# Autodesk Inventor assembly: Framing_For_Second_Floor
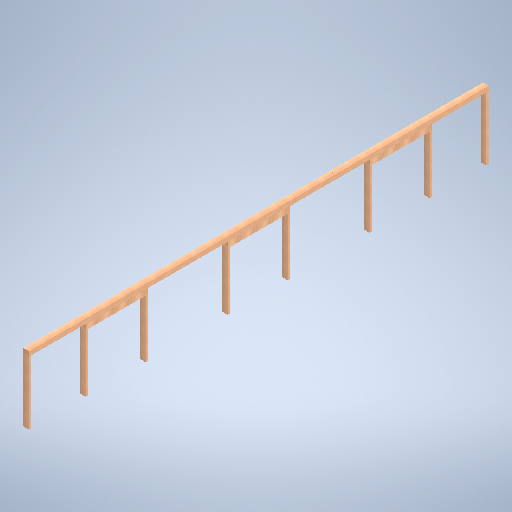
[picture p0: Inventor's stored thumbnail of the model, 512x512]
Saved by Autodesk Inventor 2025.1 (Build 291241020, 241B)
## iProperties
Created: 2024-10-21
Part Number: Framing_For_Second_Floor
Document SubType Name: Assembly
Designer: Tom
Author: Tom
## Documents named in this file (5)
- C:\Users\Tom\Documents\Inventor\Mobility\Additional_Building\Framing_For_Second_Floor.iam
- C:\Users\Tom\Documents\Inventor\Mobility\Additional_Building\Plate_With_Length_144_Inches.ipt
- C:\Users\Tom\Documents\Inventor\Mobility\Additional_Building\Plate_With_Length_96_Inches.ipt
- C:\Users\Tom\Documents\Inventor\Mobility\Additional_Building\Framing_For_Second_Floor_Window.iam
- C:\Users\Tom\Documents\Inventor\Mobility\Additional_Building\Stud_With_Height_39.5_Inches.ipt
## Components (10 placed, 4 different names)
1. Plate_With_Length_144_Inches:1 — Mate:2, Flush:3, Flush:4, Mate:3, Flush:5, Mate:4, Flush:7, Mate:9, Flush:9, Mate:12, Flush:11, Flush:12, Flush:15, Flush:16
2. Plate_With_Length_144_Inches:2 — Mate:2, Flush:3, Flush:4, Flush:6, Mate:6, Flush:8, Mate:11, Flush:10, Flush:17, Mate:13
3. Plate_With_Length_96_Inches:1 — Mate:3, Flush:5, Flush:6, Mate:5, Mate:7
4. Plate_With_Length_96_Inches:2 — Mate:4, Flush:7, Mate:5
5. Plate_With_Length_96_Inches:3 — Mate:6, Flush:8, Mate:7
6. Framing_For_Second_Floor_Window:1 [sub-assembly] — Mate:9, Flush:9, Flush:14, Flush:15
7. Framing_For_Second_Floor_Window:2 [sub-assembly] — Mate:11, Flush:10, Flush:16
8. Framing_For_Second_Floor_Window:3 [sub-assembly] — Flush:13, Flush:17, Mate:13
9. Stud_With_Height_39.5_Inches:1 — Mate:12, Flush:11, Flush:12, Flush:14
10. Stud_With_Height_39.5_Inches:2 — Flush:13
## Component patterns: (2 elements, first: Stud_With_Height_39.5_Inches:1)
## Relationships (25: Flush 15, Mate 10)
- Mate:2: Plate_With_Length_144_Inches:1 ↔ Plate_With_Length_144_Inches:2
- Flush:3: Plate_With_Length_144_Inches:1 ↔ Plate_With_Length_144_Inches:2
- Flush:4: Plate_With_Length_144_Inches:1 ↔ Plate_With_Length_144_Inches:2
- Mate:3: Plate_With_Length_144_Inches:1 ↔ Plate_With_Length_96_Inches:1
- Flush:5: Plate_With_Length_144_Inches:1 ↔ Plate_With_Length_96_Inches:1
- Flush:6 (-1219.2 mm): Plate_With_Length_144_Inches:2 ↔ Plate_With_Length_96_Inches:1
- Mate:4: Plate_With_Length_144_Inches:1 ↔ Plate_With_Length_96_Inches:2
- Flush:7: Plate_With_Length_144_Inches:1 ↔ Plate_With_Length_96_Inches:2
- Mate:5: Plate_With_Length_96_Inches:1 ↔ Plate_With_Length_96_Inches:2
- Mate:6: Plate_With_Length_144_Inches:2 ↔ Plate_With_Length_96_Inches:3
- Flush:8: Plate_With_Length_144_Inches:2 ↔ Plate_With_Length_96_Inches:3
- Mate:7: Plate_With_Length_96_Inches:1 ↔ Plate_With_Length_96_Inches:3
- Mate:9: Plate_With_Length_144_Inches:1 ↔ Framing_For_Second_Floor_Window:1
- Flush:9: Plate_With_Length_144_Inches:1 ↔ Framing_For_Second_Floor_Window:1
- Mate:11: Plate_With_Length_144_Inches:2 ↔ Framing_For_Second_Floor_Window:2
- Flush:10: Plate_With_Length_144_Inches:2 ↔ Framing_For_Second_Floor_Window:2
- Mate:12: Plate_With_Length_144_Inches:1 ↔ Stud_With_Height_39.5_Inches:1
- Flush:11: Plate_With_Length_144_Inches:1 ↔ Stud_With_Height_39.5_Inches:1
- Flush:12: Plate_With_Length_144_Inches:1 ↔ Stud_With_Height_39.5_Inches:1
- Flush:13 (-903.2875 mm): Framing_For_Second_Floor_Window:3 ↔ Stud_With_Height_39.5_Inches:2
- Flush:14 (-903.2875 mm): Framing_For_Second_Floor_Window:1 ↔ Stud_With_Height_39.5_Inches:1
- Flush:15: Plate_With_Length_144_Inches:1 ↔ Framing_For_Second_Floor_Window:1
- Flush:16: Plate_With_Length_144_Inches:1 ↔ Framing_For_Second_Floor_Window:2
- Flush:17: Plate_With_Length_144_Inches:2 ↔ Framing_For_Second_Floor_Window:3
- Mate:13: Plate_With_Length_144_Inches:2 ↔ Framing_For_Second_Floor_Window:3
